# Autodesk Inventor assembly: standing_robot_ver.1
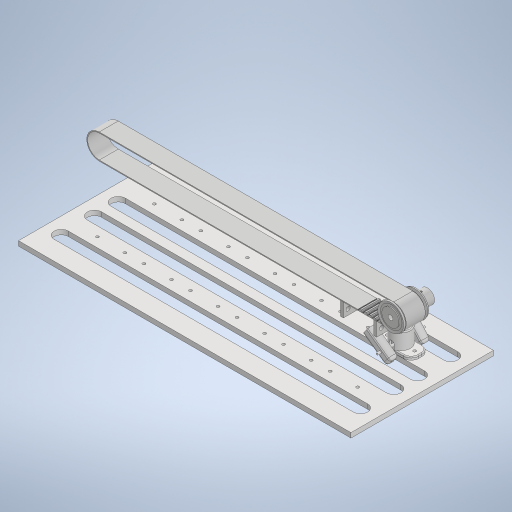
[picture p0: Inventor's stored thumbnail of the model, 512x512]
Saved by Autodesk Inventor 2023 (Build 270158000, 158)
## iProperties
Created: 2023-11-07
Part Number: standing_robot_ver.1
Document SubType Name: Assembly
Designer: bonju
Author: bonju
## Documents named in this file (8)
- C:\Users\bonju\OneDrive\デスクトップ\ikisawa\experiment8_standing\standing_robot\standing_robot_ver.1.iam
- C:\Users\bonju\OneDrive\デスクトップ\ikisawa\experiment8_standing\belt\ATBT-700T5200-B-P35_info-1-16-16.ipt
- C:\Users\bonju\OneDrive\デスクトップ\ikisawa\experiment8_standing\pulley\T5_歯数15\TTPA15T5200-B-P5_b.ipt
- C:\Users\bonju\OneDrive\デスクトップ\ikisawa\experiment8_standing\floor\floor_ver.1.ipt
- C:\Users\bonju\OneDrive\デスクトップ\ikisawa\experiment8_standing\leg_unit\cover.ver1.ipt
- C:\Users\bonju\OneDrive\デスクトップ\ikisawa\experiment8_standing\leg_unit\shaft_leg.ipt
- C:\Users\bonju\OneDrive\デスクトップ\ikisawa\experiment8_standing\leg_unit\parent_ver.1.ipt
- C:\Users\bonju\OneDrive\デスクトップ\ikisawa\experiment8_standing\leg_unit\leg.ipt
## Components (8 placed, 7 different names)
1. ATBT-700T5200-B-P35_info-1-16-16:1 — メイト:1, メイト:2, フラッシュ:1, メイト:14, フラッシュ:12
2. TTPA15T5200-B-P5_b:1 — メイト:3
3. floor_ver.1:1 — フラッシュ:11, メイト:11, メイト:12, メイト:13, メイト:14, フラッシュ:12
4. cover.ver1:1 — メイト:4, メイト:8, メイト:9, 円柱状:1, メイト:11, メイト:12, メイト:13
5. shaft_leg:1 — メイト:5, メイト:6, メイト:7, フラッシュ:2
6. parent_ver.1:1 — メイト:4, メイト:7, フラッシュ:2, 円柱状:1
7. leg:1 — メイト:5, メイト:8
8. leg:2 — メイト:6, メイト:9
## Relationships (18: Mate 13, Flush 4, CylindricalJoint 1)
- メイト:1 [Mate]: ATBT-700T5200-B-P35_info-1-16-16:1
- メイト:2 [Mate]: ATBT-700T5200-B-P35_info-1-16-16:1
- フラッシュ:1 [Flush]: ATBT-700T5200-B-P35_info-1-16-16:1
- メイト:3 [Mate]: TTPA15T5200-B-P5_b:1
- メイト:4 [Mate]: cover.ver1:1 ↔ parent_ver.1:1
- メイト:5 [Mate]: shaft_leg:1 ↔ leg:1
- メイト:6 [Mate]: shaft_leg:1 ↔ leg:2
- メイト:7 [Mate]: shaft_leg:1 ↔ parent_ver.1:1
- フラッシュ:2 [Flush]: shaft_leg:1 ↔ parent_ver.1:1
- メイト:8 [Mate] (3 mm): cover.ver1:1 ↔ leg:1
- メイト:9 [Mate] (3 mm): cover.ver1:1 ↔ leg:2
- 円柱状:1 [CylindricalJoint]: cover.ver1:1 ↔ parent_ver.1:1
- フラッシュ:11 [Flush]: floor_ver.1:1
- メイト:11 [Mate]: floor_ver.1:1 ↔ cover.ver1:1
- メイト:12 [Mate]: floor_ver.1:1 ↔ cover.ver1:1
- メイト:13 [Mate]: floor_ver.1:1 ↔ cover.ver1:1
- メイト:14 [Mate] (50 mm): ATBT-700T5200-B-P35_info-1-16-16:1 ↔ floor_ver.1:1
- フラッシュ:12 [Flush]: ATBT-700T5200-B-P35_info-1-16-16:1 ↔ floor_ver.1:1
